# Autodesk Inventor assembly: front_box
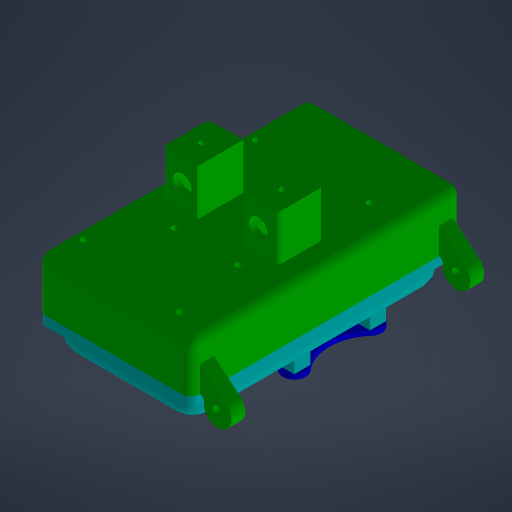
[picture p0: Inventor's stored thumbnail of the model, 512x512]
Saved by Autodesk Inventor 2024 (Build 280153000, 153)
## iProperties
Created: 2023-05-12
Part Number: front_box
Document SubType Name: Assembly
Designer: user
Author: user
## Documents named in this file (6)
- D:\Docs\Robot\3d\machine_body\front_box_asembly.iam
- D:\Docs\Robot\3d\machine_body\front_box_asembly\front_box.ipt
- D:\Docs\Robot\3d\electronics\Arduino MEGA 2560 R3.ipt
- D:\Docs\Robot\3d\electronics\ts832.ipt
- D:\Docs\Robot\3d\machine_body\front_box_asembly\ts_holder.ipt
- D:\Docs\Robot\3d\machine_body\front_box_asembly\front_box_cup.ipt
## Components (5 placed, 5 different names)
1. front_box:1 — Совмещение:1, Заподлицо:1, Совмещение:3, Совмещение:4, Совмещение:5, Совмещение:6, Совмещение:7, Совмещение:8, Совмещение:9
2. Arduino MEGA 2560 R3:1 — Совмещение:3, Совмещение:4, Совмещение:5
3. ts832:1 — Совмещение:10, Совмещение:11, Совмещение:12
4. ts_holder:1 — Вставка:1, Вставка:2
5. front_box_cup:1 — Совмещение:7, Совмещение:8, Совмещение:9, Совмещение:10, Совмещение:11, Совмещение:12, Вставка:1, Вставка:2
## Relationships (14: Mate 11, Insert 2, Flush 1)
- Совмещение:1 [Mate]: front_box:1
- Заподлицо:1 [Flush]: front_box:1
- Совмещение:3 [Mate]: front_box:1 ↔ Arduino MEGA 2560 R3:1
- Совмещение:4 [Mate]: front_box:1 ↔ Arduino MEGA 2560 R3:1
- Совмещение:5 [Mate]: front_box:1 ↔ Arduino MEGA 2560 R3:1
- Совмещение:6 [Mate]: front_box:1
- Совмещение:7 [Mate]: front_box:1 ↔ front_box_cup:1
- Совмещение:8 [Mate]: front_box:1 ↔ front_box_cup:1
- Совмещение:9 [Mate]: front_box:1 ↔ front_box_cup:1
- Совмещение:10 [Mate]: ts832:1 ↔ front_box_cup:1
- Совмещение:11 [Mate]: ts832:1 ↔ front_box_cup:1
- Совмещение:12 [Mate]: ts832:1 ↔ front_box_cup:1
- Вставка:1 [Insert]: ts_holder:1 ↔ front_box_cup:1
- Вставка:2 [Insert]: ts_holder:1 ↔ front_box_cup:1
